(part 1 of 3)
# Autodesk Inventor assembly: HDR_2.54mm_RGB4078660_1
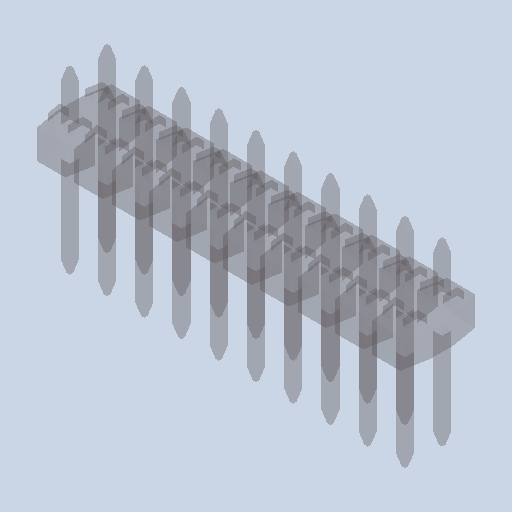
[picture p0: Inventor's stored thumbnail of the model, 512x512]
Saved by Autodesk Inventor 2026 (Build 300175050, 175E)
## iProperties
Created: 2025-07-29
Part Number: HDR_2.54mm_RGB4078660_1
Document SubType Name: Assembly
Designer: tdxt
Author: tdxt
## Documents named in this file (625)
- D:\Github\Pandoras_Box\CAD\pandoras_box_R2\pandoras_box_R2\HDR_2.54mm_RGB4078660_1.iam
- D:\Github\Pandoras_Box\CAD\pandoras_box_R2\pandoras_box_R2\Open CASCADE STEP translator 6.8 1.452.1.1.ipt
- D:\Github\Pandoras_Box\CAD\pandoras_box_R2\pandoras_box_R2\Open CASCADE STEP translator 6.8 1.452.1.2.ipt
- D:\Github\Pandoras_Box\CAD\pandoras_box_R2\pandoras_box_R2\Open CASCADE STEP translator 6.8 1.452.1.3.ipt
- D:\Github\Pandoras_Box\CAD\pandoras_box_R2\pandoras_box_R2\Open CASCADE STEP translator 6.8 1.452.1.4.ipt
- D:\Github\Pandoras_Box\CAD\pandoras_box_R2\pandoras_box_R2\Open CASCADE STEP translator 6.8 1.452.1.5.ipt
- D:\Github\Pandoras_Box\CAD\pandoras_box_R2\pandoras_box_R2\Open CASCADE STEP translator 6.8 1.452.1.6.ipt
- D:\Github\Pandoras_Box\CAD\pandoras_box_R2\pandoras_box_R2\Open CASCADE STEP translator 6.8 1.452.1.7.ipt
- D:\Github\Pandoras_Box\CAD\pandoras_box_R2\pandoras_box_R2\Open CASCADE STEP translator 6.8 1.452.1.8.ipt
- D:\Github\Pandoras_Box\CAD\pandoras_box_R2\pandoras_box_R2\Open CASCADE STEP translator 6.8 1.452.1.9.ipt
- D:\Github\Pandoras_Box\CAD\pandoras_box_R2\pandoras_box_R2\Open CASCADE STEP translator 6.8 1.452.1.10.ipt
- D:\Github\Pandoras_Box\CAD\pandoras_box_R2\pandoras_box_R2\Open CASCADE STEP translator 6.8 1.452.1.11.ipt
- D:\Github\Pandoras_Box\CAD\pandoras_box_R2\pandoras_box_R2\Open CASCADE STEP translator 6.8 1.452.1.12.ipt
- D:\Github\Pandoras_Box\CAD\pandoras_box_R2\pandoras_box_R2\Open CASCADE STEP translator 6.8 1.452.1.13.ipt
- D:\Github\Pandoras_Box\CAD\pandoras_box_R2\pandoras_box_R2\Open CASCADE STEP translator 6.8 1.452.1.14.ipt
- D:\Github\Pandoras_Box\CAD\pandoras_box_R2\pandoras_box_R2\Open CASCADE STEP translator 6.8 1.452.1.15.ipt
- D:\Github\Pandoras_Box\CAD\pandoras_box_R2\pandoras_box_R2\Open CASCADE STEP translator 6.8 1.452.1.16.ipt
- D:\Github\Pandoras_Box\CAD\pandoras_box_R2\pandoras_box_R2\Open CASCADE STEP translator 6.8 1.452.1.17.ipt
- D:\Github\Pandoras_Box\CAD\pandoras_box_R2\pandoras_box_R2\Open CASCADE STEP translator 6.8 1.452.1.18.ipt
- D:\Github\Pandoras_Box\CAD\pandoras_box_R2\pandoras_box_R2\Open CASCADE STEP translator 6.8 1.452.1.19.ipt
- D:\Github\Pandoras_Box\CAD\pandoras_box_R2\pandoras_box_R2\Open CASCADE STEP translator 6.8 1.452.1.20.ipt
- D:\Github\Pandoras_Box\CAD\pandoras_box_R2\pandoras_box_R2\Open CASCADE STEP translator 6.8 1.452.1.21.ipt
- D:\Github\Pandoras_Box\CAD\pandoras_box_R2\pandoras_box_R2\Open CASCADE STEP translator 6.8 1.452.1.22.ipt
- D:\Github\Pandoras_Box\CAD\pandoras_box_R2\pandoras_box_R2\Open CASCADE STEP translator 6.8 1.452.1.23.ipt
- D:\Github\Pandoras_Box\CAD\pandoras_box_R2\pandoras_box_R2\Open CASCADE STEP translator 6.8 1.452.1.24.ipt
- D:\Github\Pandoras_Box\CAD\pandoras_box_R2\pandoras_box_R2\Open CASCADE STEP translator 6.8 1.452.1.25.ipt
- D:\Github\Pandoras_Box\CAD\pandoras_box_R2\pandoras_box_R2\Open CASCADE STEP translator 6.8 1.452.1.26.ipt
- D:\Github\Pandoras_Box\CAD\pandoras_box_R2\pandoras_box_R2\Open CASCADE STEP translator 6.8 1.452.1.27.ipt
- D:\Github\Pandoras_Box\CAD\pandoras_box_R2\pandoras_box_R2\Open CASCADE STEP translator 6.8 1.452.1.28.ipt
- D:\Github\Pandoras_Box\CAD\pandoras_box_R2\pandoras_box_R2\Open CASCADE STEP translator 6.8 1.452.1.29.ipt
- D:\Github\Pandoras_Box\CAD\pandoras_box_R2\pandoras_box_R2\Open CASCADE STEP translator 6.8 1.452.1.30.ipt
- D:\Github\Pandoras_Box\CAD\pandoras_box_R2\pandoras_box_R2\Open CASCADE STEP translator 6.8 1.452.1.31.ipt
- D:\Github\Pandoras_Box\CAD\pandoras_box_R2\pandoras_box_R2\Open CASCADE STEP translator 6.8 1.452.1.32.ipt
- D:\Github\Pandoras_Box\CAD\pandoras_box_R2\pandoras_box_R2\Open CASCADE STEP translator 6.8 1.452.1.33.ipt
- D:\Github\Pandoras_Box\CAD\pandoras_box_R2\pandoras_box_R2\Open CASCADE STEP translator 6.8 1.452.1.34.ipt
- D:\Github\Pandoras_Box\CAD\pandoras_box_R2\pandoras_box_R2\Open CASCADE STEP translator 6.8 1.452.1.35.ipt
- D:\Github\Pandoras_Box\CAD\pandoras_box_R2\pandoras_box_R2\Open CASCADE STEP translator 6.8 1.452.1.36.ipt
- D:\Github\Pandoras_Box\CAD\pandoras_box_R2\pandoras_box_R2\Open CASCADE STEP translator 6.8 1.452.1.37.ipt
- D:\Github\Pandoras_Box\CAD\pandoras_box_R2\pandoras_box_R2\Open CASCADE STEP translator 6.8 1.452.1.38.ipt
- D:\Github\Pandoras_Box\CAD\pandoras_box_R2\pandoras_box_R2\Open CASCADE STEP translator 6.8 1.452.1.39.ipt
- D:\Github\Pandoras_Box\CAD\pandoras_box_R2\pandoras_box_R2\Open CASCADE STEP translator 6.8 1.452.1.40.ipt
- D:\Github\Pandoras_Box\CAD\pandoras_box_R2\pandoras_box_R2\Open CASCADE STEP translator 6.8 1.452.1.41.ipt
- D:\Github\Pandoras_Box\CAD\pandoras_box_R2\pandoras_box_R2\Open CASCADE STEP translator 6.8 1.452.1.42.ipt
- D:\Github\Pandoras_Box\CAD\pandoras_box_R2\pandoras_box_R2\Open CASCADE STEP translator 6.8 1.452.1.43.ipt
- D:\Github\Pandoras_Box\CAD\pandoras_box_R2\pandoras_box_R2\Open CASCADE STEP translator 6.8 1.452.1.44.ipt
- D:\Github\Pandoras_Box\CAD\pandoras_box_R2\pandoras_box_R2\Open CASCADE STEP translator 6.8 1.452.1.45.ipt
- D:\Github\Pandoras_Box\CAD\pandoras_box_R2\pandoras_box_R2\Open CASCADE STEP translator 6.8 1.452.1.46.ipt
- D:\Github\Pandoras_Box\CAD\pandoras_box_R2\pandoras_box_R2\Open CASCADE STEP translator 6.8 1.452.1.47.ipt
- D:\Github\Pandoras_Box\CAD\pandoras_box_R2\pandoras_box_R2\Open CASCADE STEP translator 6.8 1.452.1.48.ipt
- D:\Github\Pandoras_Box\CAD\pandoras_box_R2\pandoras_box_R2\Open CASCADE STEP translator 6.8 1.452.1.49.ipt
- D:\Github\Pandoras_Box\CAD\pandoras_box_R2\pandoras_box_R2\Open CASCADE STEP translator 6.8 1.452.1.50.ipt
- D:\Github\Pandoras_Box\CAD\pandoras_box_R2\pandoras_box_R2\Open CASCADE STEP translator 6.8 1.452.1.51.ipt
- D:\Github\Pandoras_Box\CAD\pandoras_box_R2\pandoras_box_R2\Open CASCADE STEP translator 6.8 1.452.1.52.ipt
- D:\Github\Pandoras_Box\CAD\pandoras_box_R2\pandoras_box_R2\Open CASCADE STEP translator 6.8 1.452.1.53.ipt
- D:\Github\Pandoras_Box\CAD\pandoras_box_R2\pandoras_box_R2\Open CASCADE STEP translator 6.8 1.452.1.54.ipt
- D:\Github\Pandoras_Box\CAD\pandoras_box_R2\pandoras_box_R2\Open CASCADE STEP translator 6.8 1.452.1.55.ipt
- D:\Github\Pandoras_Box\CAD\pandoras_box_R2\pandoras_box_R2\Open CASCADE STEP translator 6.8 1.452.1.56.ipt
- D:\Github\Pandoras_Box\CAD\pandoras_box_R2\pandoras_box_R2\Open CASCADE STEP translator 6.8 1.452.1.57.ipt
- D:\Github\Pandoras_Box\CAD\pandoras_box_R2\pandoras_box_R2\Open CASCADE STEP translator 6.8 1.452.1.58.ipt
- D:\Github\Pandoras_Box\CAD\pandoras_box_R2\pandoras_box_R2\Open CASCADE STEP translator 6.8 1.452.1.59.ipt
- D:\Github\Pandoras_Box\CAD\pandoras_box_R2\pandoras_box_R2\Open CASCADE STEP translator 6.8 1.452.1.60.ipt
- D:\Github\Pandoras_Box\CAD\pandoras_box_R2\pandoras_box_R2\Open CASCADE STEP translator 6.8 1.452.1.61.ipt
- D:\Github\Pandoras_Box\CAD\pandoras_box_R2\pandoras_box_R2\Open CASCADE STEP translator 6.8 1.452.1.62.ipt
- D:\Github\Pandoras_Box\CAD\pandoras_box_R2\pandoras_box_R2\Open CASCADE STEP translator 6.8 1.452.1.63.ipt
- D:\Github\Pandoras_Box\CAD\pandoras_box_R2\pandoras_box_R2\Open CASCADE STEP translator 6.8 1.452.1.64.ipt
- D:\Github\Pandoras_Box\CAD\pandoras_box_R2\pandoras_box_R2\Open CASCADE STEP translator 6.8 1.452.1.65.ipt
- D:\Github\Pandoras_Box\CAD\pandoras_box_R2\pandoras_box_R2\Open CASCADE STEP translator 6.8 1.452.1.66.ipt
- D:\Github\Pandoras_Box\CAD\pandoras_box_R2\pandoras_box_R2\Open CASCADE STEP translator 6.8 1.452.1.67.ipt
- D:\Github\Pandoras_Box\CAD\pandoras_box_R2\pandoras_box_R2\Open CASCADE STEP translator 6.8 1.452.1.68.ipt
- D:\Github\Pandoras_Box\CAD\pandoras_box_R2\pandoras_box_R2\Open CASCADE STEP translator 6.8 1.452.1.69.ipt
- D:\Github\Pandoras_Box\CAD\pandoras_box_R2\pandoras_box_R2\Open CASCADE STEP translator 6.8 1.452.1.70.ipt
- D:\Github\Pandoras_Box\CAD\pandoras_box_R2\pandoras_box_R2\Open CASCADE STEP translator 6.8 1.452.1.71.ipt
- D:\Github\Pandoras_Box\CAD\pandoras_box_R2\pandoras_box_R2\Open CASCADE STEP translator 6.8 1.452.1.72.ipt
- D:\Github\Pandoras_Box\CAD\pandoras_box_R2\pandoras_box_R2\Open CASCADE STEP translator 6.8 1.452.1.73.ipt
- D:\Github\Pandoras_Box\CAD\pandoras_box_R2\pandoras_box_R2\Open CASCADE STEP translator 6.8 1.452.1.74.ipt
- D:\Github\Pandoras_Box\CAD\pandoras_box_R2\pandoras_box_R2\Open CASCADE STEP translator 6.8 1.452.1.75.ipt
- D:\Github\Pandoras_Box\CAD\pandoras_box_R2\pandoras_box_R2\Open CASCADE STEP translator 6.8 1.452.1.76.ipt
- D:\Github\Pandoras_Box\CAD\pandoras_box_R2\pandoras_box_R2\Open CASCADE STEP translator 6.8 1.452.1.77.ipt
- D:\Github\Pandoras_Box\CAD\pandoras_box_R2\pandoras_box_R2\Open CASCADE STEP translator 6.8 1.452.1.78.ipt
- D:\Github\Pandoras_Box\CAD\pandoras_box_R2\pandoras_box_R2\Open CASCADE STEP translator 6.8 1.452.1.79.ipt
- D:\Github\Pandoras_Box\CAD\pandoras_box_R2\pandoras_box_R2\Open CASCADE STEP translator 6.8 1.452.1.80.ipt
- D:\Github\Pandoras_Box\CAD\pandoras_box_R2\pandoras_box_R2\Open CASCADE STEP translator 6.8 1.452.1.81.ipt
- D:\Github\Pandoras_Box\CAD\pandoras_box_R2\pandoras_box_R2\Open CASCADE STEP translator 6.8 1.452.1.82.ipt
- D:\Github\Pandoras_Box\CAD\pandoras_box_R2\pandoras_box_R2\Open CASCADE STEP translator 6.8 1.452.1.83.ipt
- D:\Github\Pandoras_Box\CAD\pandoras_box_R2\pandoras_box_R2\Open CASCADE STEP translator 6.8 1.452.1.84.ipt
- D:\Github\Pandoras_Box\CAD\pandoras_box_R2\pandoras_box_R2\Open CASCADE STEP translator 6.8 1.452.1.85.ipt
- D:\Github\Pandoras_Box\CAD\pandoras_box_R2\pandoras_box_R2\Open CASCADE STEP translator 6.8 1.452.1.86.ipt
- D:\Github\Pandoras_Box\CAD\pandoras_box_R2\pandoras_box_R2\Open CASCADE STEP translator 6.8 1.452.1.87.ipt
- D:\Github\Pandoras_Box\CAD\pandoras_box_R2\pandoras_box_R2\Open CASCADE STEP translator 6.8 1.452.1.88.ipt
- D:\Github\Pandoras_Box\CAD\pandoras_box_R2\pandoras_box_R2\Open CASCADE STEP translator 6.8 1.452.1.89.ipt
- D:\Github\Pandoras_Box\CAD\pandoras_box_R2\pandoras_box_R2\Open CASCADE STEP translator 6.8 1.452.1.90.ipt
- D:\Github\Pandoras_Box\CAD\pandoras_box_R2\pandoras_box_R2\Open CASCADE STEP translator 6.8 1.452.1.91.ipt
- D:\Github\Pandoras_Box\CAD\pandoras_box_R2\pandoras_box_R2\Open CASCADE STEP translator 6.8 1.452.1.92.ipt
- D:\Github\Pandoras_Box\CAD\pandoras_box_R2\pandoras_box_R2\Open CASCADE STEP translator 6.8 1.452.1.93.ipt
- D:\Github\Pandoras_Box\CAD\pandoras_box_R2\pandoras_box_R2\Open CASCADE STEP translator 6.8 1.452.1.94.ipt
- D:\Github\Pandoras_Box\CAD\pandoras_box_R2\pandoras_box_R2\Open CASCADE STEP translator 6.8 1.452.1.95.ipt
- D:\Github\Pandoras_Box\CAD\pandoras_box_R2\pandoras_box_R2\Open CASCADE STEP translator 6.8 1.452.1.96.ipt
- D:\Github\Pandoras_Box\CAD\pandoras_box_R2\pandoras_box_R2\Open CASCADE STEP translator 6.8 1.452.1.97.ipt
- D:\Github\Pandoras_Box\CAD\pandoras_box_R2\pandoras_box_R2\Open CASCADE STEP translator 6.8 1.452.1.98.ipt
- D:\Github\Pandoras_Box\CAD\pandoras_box_R2\pandoras_box_R2\Open CASCADE STEP translator 6.8 1.452.1.99.ipt
- D:\Github\Pandoras_Box\CAD\pandoras_box_R2\pandoras_box_R2\Open CASCADE STEP translator 6.8 1.452.1.100.ipt
- D:\Github\Pandoras_Box\CAD\pandoras_box_R2\pandoras_box_R2\Open CASCADE STEP translator 6.8 1.452.1.101.ipt
- D:\Github\Pandoras_Box\CAD\pandoras_box_R2\pandoras_box_R2\Open CASCADE STEP translator 6.8 1.452.1.102.ipt
- D:\Github\Pandoras_Box\CAD\pandoras_box_R2\pandoras_box_R2\Open CASCADE STEP translator 6.8 1.452.1.103.ipt
- D:\Github\Pandoras_Box\CAD\pandoras_box_R2\pandoras_box_R2\Open CASCADE STEP translator 6.8 1.452.1.104.ipt
- D:\Github\Pandoras_Box\CAD\pandoras_box_R2\pandoras_box_R2\Open CASCADE STEP translator 6.8 1.452.1.105.ipt
- D:\Github\Pandoras_Box\CAD\pandoras_box_R2\pandoras_box_R2\Open CASCADE STEP translator 6.8 1.452.1.106.ipt
- D:\Github\Pandoras_Box\CAD\pandoras_box_R2\pandoras_box_R2\Open CASCADE STEP translator 6.8 1.452.1.107.ipt
- D:\Github\Pandoras_Box\CAD\pandoras_box_R2\pandoras_box_R2\Open CASCADE STEP translator 6.8 1.452.1.108.ipt
- D:\Github\Pandoras_Box\CAD\pandoras_box_R2\pandoras_box_R2\Open CASCADE STEP translator 6.8 1.452.1.109.ipt
- D:\Github\Pandoras_Box\CAD\pandoras_box_R2\pandoras_box_R2\Open CASCADE STEP translator 6.8 1.452.1.110.ipt
- D:\Github\Pandoras_Box\CAD\pandoras_box_R2\pandoras_box_R2\Open CASCADE STEP translator 6.8 1.452.1.111.ipt
- D:\Github\Pandoras_Box\CAD\pandoras_box_R2\pandoras_box_R2\Open CASCADE STEP translator 6.8 1.452.1.112.ipt
- D:\Github\Pandoras_Box\CAD\pandoras_box_R2\pandoras_box_R2\Open CASCADE STEP translator 6.8 1.452.1.113.ipt
- D:\Github\Pandoras_Box\CAD\pandoras_box_R2\pandoras_box_R2\Open CASCADE STEP translator 6.8 1.452.1.114.ipt
- D:\Github\Pandoras_Box\CAD\pandoras_box_R2\pandoras_box_R2\Open CASCADE STEP translator 6.8 1.452.1.115.ipt
- D:\Github\Pandoras_Box\CAD\pandoras_box_R2\pandoras_box_R2\Open CASCADE STEP translator 6.8 1.452.1.116.ipt
- D:\Github\Pandoras_Box\CAD\pandoras_box_R2\pandoras_box_R2\Open CASCADE STEP translator 6.8 1.452.1.117.ipt
- D:\Github\Pandoras_Box\CAD\pandoras_box_R2\pandoras_box_R2\Open CASCADE STEP translator 6.8 1.452.1.118.ipt
- D:\Github\Pandoras_Box\CAD\pandoras_box_R2\pandoras_box_R2\Open CASCADE STEP translator 6.8 1.452.1.119.ipt
- D:\Github\Pandoras_Box\CAD\pandoras_box_R2\pandoras_box_R2\Open CASCADE STEP translator 6.8 1.452.1.120.ipt
- D:\Github\Pandoras_Box\CAD\pandoras_box_R2\pandoras_box_R2\Open CASCADE STEP translator 6.8 1.452.1.121.ipt
- D:\Github\Pandoras_Box\CAD\pandoras_box_R2\pandoras_box_R2\Open CASCADE STEP translator 6.8 1.452.1.122.ipt
- D:\Github\Pandoras_Box\CAD\pandoras_box_R2\pandoras_box_R2\Open CASCADE STEP translator 6.8 1.452.1.123.ipt
- D:\Github\Pandoras_Box\CAD\pandoras_box_R2\pandoras_box_R2\Open CASCADE STEP translator 6.8 1.452.1.124.ipt
- D:\Github\Pandoras_Box\CAD\pandoras_box_R2\pandoras_box_R2\Open CASCADE STEP translator 6.8 1.452.1.125.ipt
- D:\Github\Pandoras_Box\CAD\pandoras_box_R2\pandoras_box_R2\Open CASCADE STEP translator 6.8 1.452.1.126.ipt
- D:\Github\Pandoras_Box\CAD\pandoras_box_R2\pandoras_box_R2\Open CASCADE STEP translator 6.8 1.452.1.127.ipt
- D:\Github\Pandoras_Box\CAD\pandoras_box_R2\pandoras_box_R2\Open CASCADE STEP translator 6.8 1.452.1.128.ipt
- D:\Github\Pandoras_Box\CAD\pandoras_box_R2\pandoras_box_R2\Open CASCADE STEP translator 6.8 1.452.1.129.ipt
- D:\Github\Pandoras_Box\CAD\pandoras_box_R2\pandoras_box_R2\Open CASCADE STEP translator 6.8 1.452.1.130.ipt
- D:\Github\Pandoras_Box\CAD\pandoras_box_R2\pandoras_box_R2\Open CASCADE STEP translator 6.8 1.452.1.131.ipt
- D:\Github\Pandoras_Box\CAD\pandoras_box_R2\pandoras_box_R2\Open CASCADE STEP translator 6.8 1.452.1.132.ipt
- D:\Github\Pandoras_Box\CAD\pandoras_box_R2\pandoras_box_R2\Open CASCADE STEP translator 6.8 1.452.1.133.ipt
- D:\Github\Pandoras_Box\CAD\pandoras_box_R2\pandoras_box_R2\Open CASCADE STEP translator 6.8 1.452.1.134.ipt
- D:\Github\Pandoras_Box\CAD\pandoras_box_R2\pandoras_box_R2\Open CASCADE STEP translator 6.8 1.452.1.135.ipt
- D:\Github\Pandoras_Box\CAD\pandoras_box_R2\pandoras_box_R2\Open CASCADE STEP translator 6.8 1.452.1.136.ipt
- D:\Github\Pandoras_Box\CAD\pandoras_box_R2\pandoras_box_R2\Open CASCADE STEP translator 6.8 1.452.1.137.ipt
- D:\Github\Pandoras_Box\CAD\pandoras_box_R2\pandoras_box_R2\Open CASCADE STEP translator 6.8 1.452.1.138.ipt
- D:\Github\Pandoras_Box\CAD\pandoras_box_R2\pandoras_box_R2\Open CASCADE STEP translator 6.8 1.452.1.139.ipt
- D:\Github\Pandoras_Box\CAD\pandoras_box_R2\pandoras_box_R2\Open CASCADE STEP translator 6.8 1.452.1.140.ipt
- D:\Github\Pandoras_Box\CAD\pandoras_box_R2\pandoras_box_R2\Open CASCADE STEP translator 6.8 1.452.1.141.ipt
- D:\Github\Pandoras_Box\CAD\pandoras_box_R2\pandoras_box_R2\Open CASCADE STEP translator 6.8 1.452.1.142.ipt
- D:\Github\Pandoras_Box\CAD\pandoras_box_R2\pandoras_box_R2\Open CASCADE STEP translator 6.8 1.452.1.143.ipt
- D:\Github\Pandoras_Box\CAD\pandoras_box_R2\pandoras_box_R2\Open CASCADE STEP translator 6.8 1.452.1.144.ipt
- D:\Github\Pandoras_Box\CAD\pandoras_box_R2\pandoras_box_R2\Open CASCADE STEP translator 6.8 1.452.1.145.ipt
- D:\Github\Pandoras_Box\CAD\pandoras_box_R2\pandoras_box_R2\Open CASCADE STEP translator 6.8 1.452.1.146.ipt
- D:\Github\Pandoras_Box\CAD\pandoras_box_R2\pandoras_box_R2\Open CASCADE STEP translator 6.8 1.452.1.147.ipt
- D:\Github\Pandoras_Box\CAD\pandoras_box_R2\pandoras_box_R2\Open CASCADE STEP translator 6.8 1.452.1.148.ipt
- D:\Github\Pandoras_Box\CAD\pandoras_box_R2\pandoras_box_R2\Open CASCADE STEP translator 6.8 1.452.1.149.ipt
- D:\Github\Pandoras_Box\CAD\pandoras_box_R2\pandoras_box_R2\Open CASCADE STEP translator 6.8 1.452.1.150.ipt
- D:\Github\Pandoras_Box\CAD\pandoras_box_R2\pandoras_box_R2\Open CASCADE STEP translator 6.8 1.452.1.151.ipt
- D:\Github\Pandoras_Box\CAD\pandoras_box_R2\pandoras_box_R2\Open CASCADE STEP translator 6.8 1.452.1.152.ipt
- D:\Github\Pandoras_Box\CAD\pandoras_box_R2\pandoras_box_R2\Open CASCADE STEP translator 6.8 1.452.1.153.ipt
- D:\Github\Pandoras_Box\CAD\pandoras_box_R2\pandoras_box_R2\Open CASCADE STEP translator 6.8 1.452.1.154.ipt
- D:\Github\Pandoras_Box\CAD\pandoras_box_R2\pandoras_box_R2\Open CASCADE STEP translator 6.8 1.452.1.155.ipt
- D:\Github\Pandoras_Box\CAD\pandoras_box_R2\pandoras_box_R2\Open CASCADE STEP translator 6.8 1.452.1.156.ipt
- D:\Github\Pandoras_Box\CAD\pandoras_box_R2\pandoras_box_R2\Open CASCADE STEP translator 6.8 1.452.1.157.ipt
- D:\Github\Pandoras_Box\CAD\pandoras_box_R2\pandoras_box_R2\Open CASCADE STEP translator 6.8 1.452.1.158.ipt
- D:\Github\Pandoras_Box\CAD\pandoras_box_R2\pandoras_box_R2\Open CASCADE STEP translator 6.8 1.452.1.159.ipt
- D:\Github\Pandoras_Box\CAD\pandoras_box_R2\pandoras_box_R2\Open CASCADE STEP translator 6.8 1.452.1.160.ipt
- D:\Github\Pandoras_Box\CAD\pandoras_box_R2\pandoras_box_R2\Open CASCADE STEP translator 6.8 1.452.1.161.ipt
- D:\Github\Pandoras_Box\CAD\pandoras_box_R2\pandoras_box_R2\Open CASCADE STEP translator 6.8 1.452.1.162.ipt
- D:\Github\Pandoras_Box\CAD\pandoras_box_R2\pandoras_box_R2\Open CASCADE STEP translator 6.8 1.452.1.163.ipt
- D:\Github\Pandoras_Box\CAD\pandoras_box_R2\pandoras_box_R2\Open CASCADE STEP translator 6.8 1.452.1.164.ipt
- D:\Github\Pandoras_Box\CAD\pandoras_box_R2\pandoras_box_R2\Open CASCADE STEP translator 6.8 1.452.1.165.ipt
- D:\Github\Pandoras_Box\CAD\pandoras_box_R2\pandoras_box_R2\Open CASCADE STEP translator 6.8 1.452.1.166.ipt
- D:\Github\Pandoras_Box\CAD\pandoras_box_R2\pandoras_box_R2\Open CASCADE STEP translator 6.8 1.452.1.167.ipt
- D:\Github\Pandoras_Box\CAD\pandoras_box_R2\pandoras_box_R2\Open CASCADE STEP translator 6.8 1.452.1.168.ipt
- D:\Github\Pandoras_Box\CAD\pandoras_box_R2\pandoras_box_R2\Open CASCADE STEP translator 6.8 1.452.1.169.ipt
- D:\Github\Pandoras_Box\CAD\pandoras_box_R2\pandoras_box_R2\Open CASCADE STEP translator 6.8 1.452.1.170.ipt
- D:\Github\Pandoras_Box\CAD\pandoras_box_R2\pandoras_box_R2\Open CASCADE STEP translator 6.8 1.452.1.171.ipt
- D:\Github\Pandoras_Box\CAD\pandoras_box_R2\pandoras_box_R2\Open CASCADE STEP translator 6.8 1.452.1.172.ipt
- D:\Github\Pandoras_Box\CAD\pandoras_box_R2\pandoras_box_R2\Open CASCADE STEP translator 6.8 1.452.1.173.ipt
- D:\Github\Pandoras_Box\CAD\pandoras_box_R2\pandoras_box_R2\Open CASCADE STEP translator 6.8 1.452.1.174.ipt
- D:\Github\Pandoras_Box\CAD\pandoras_box_R2\pandoras_box_R2\Open CASCADE STEP translator 6.8 1.452.1.175.ipt
- D:\Github\Pandoras_Box\CAD\pandoras_box_R2\pandoras_box_R2\Open CASCADE STEP translator 6.8 1.452.1.176.ipt
- D:\Github\Pandoras_Box\CAD\pandoras_box_R2\pandoras_box_R2\Open CASCADE STEP translator 6.8 1.452.1.177.ipt
- D:\Github\Pandoras_Box\CAD\pandoras_box_R2\pandoras_box_R2\Open CASCADE STEP translator 6.8 1.452.1.178.ipt
- D:\Github\Pandoras_Box\CAD\pandoras_box_R2\pandoras_box_R2\Open CASCADE STEP translator 6.8 1.452.1.179.ipt
- D:\Github\Pandoras_Box\CAD\pandoras_box_R2\pandoras_box_R2\Open CASCADE STEP translator 6.8 1.452.1.180.ipt
- D:\Github\Pandoras_Box\CAD\pandoras_box_R2\pandoras_box_R2\Open CASCADE STEP translator 6.8 1.452.1.181.ipt
- D:\Github\Pandoras_Box\CAD\pandoras_box_R2\pandoras_box_R2\Open CASCADE STEP translator 6.8 1.452.1.182.ipt
- D:\Github\Pandoras_Box\CAD\pandoras_box_R2\pandoras_box_R2\Open CASCADE STEP translator 6.8 1.452.1.183.ipt
- D:\Github\Pandoras_Box\CAD\pandoras_box_R2\pandoras_box_R2\Open CASCADE STEP translator 6.8 1.452.1.184.ipt
- D:\Github\Pandoras_Box\CAD\pandoras_box_R2\pandoras_box_R2\Open CASCADE STEP translator 6.8 1.452.1.185.ipt
- D:\Github\Pandoras_Box\CAD\pandoras_box_R2\pandoras_box_R2\Open CASCADE STEP translator 6.8 1.452.1.186.ipt
- D:\Github\Pandoras_Box\CAD\pandoras_box_R2\pandoras_box_R2\Open CASCADE STEP translator 6.8 1.452.1.187.ipt
- D:\Github\Pandoras_Box\CAD\pandoras_box_R2\pandoras_box_R2\Open CASCADE STEP translator 6.8 1.452.1.188.ipt
- D:\Github\Pandoras_Box\CAD\pandoras_box_R2\pandoras_box_R2\Open CASCADE STEP translator 6.8 1.452.1.189.ipt
- D:\Github\Pandoras_Box\CAD\pandoras_box_R2\pandoras_box_R2\Open CASCADE STEP translator 6.8 1.452.1.190.ipt
- D:\Github\Pandoras_Box\CAD\pandoras_box_R2\pandoras_box_R2\Open CASCADE STEP translator 6.8 1.452.1.191.ipt
- D:\Github\Pandoras_Box\CAD\pandoras_box_R2\pandoras_box_R2\Open CASCADE STEP translator 6.8 1.452.1.192.ipt
- D:\Github\Pandoras_Box\CAD\pandoras_box_R2\pandoras_box_R2\Open CASCADE STEP translator 6.8 1.452.1.193.ipt
- D:\Github\Pandoras_Box\CAD\pandoras_box_R2\pandoras_box_R2\Open CASCADE STEP translator 6.8 1.452.1.194.ipt
- D:\Github\Pandoras_Box\CAD\pandoras_box_R2\pandoras_box_R2\Open CASCADE STEP translator 6.8 1.452.1.195.ipt
- D:\Github\Pandoras_Box\CAD\pandoras_box_R2\pandoras_box_R2\Open CASCADE STEP translator 6.8 1.452.1.196.ipt
- D:\Github\Pandoras_Box\CAD\pandoras_box_R2\pandoras_box_R2\Open CASCADE STEP translator 6.8 1.452.1.197.ipt
- D:\Github\Pandoras_Box\CAD\pandoras_box_R2\pandoras_box_R2\Open CASCADE STEP translator 6.8 1.452.1.198.ipt
- D:\Github\Pandoras_Box\CAD\pandoras_box_R2\pandoras_box_R2\Open CASCADE STEP translator 6.8 1.452.1.199.ipt
- D:\Github\Pandoras_Box\CAD\pandoras_box_R2\pandoras_box_R2\Open CASCADE STEP translator 6.8 1.452.1.200.ipt
- D:\Github\Pandoras_Box\CAD\pandoras_box_R2\pandoras_box_R2\Open CASCADE STEP translator 6.8 1.452.1.201.ipt
- D:\Github\Pandoras_Box\CAD\pandoras_box_R2\pandoras_box_R2\Open CASCADE STEP translator 6.8 1.452.1.202.ipt
- D:\Github\Pandoras_Box\CAD\pandoras_box_R2\pandoras_box_R2\Open CASCADE STEP translator 6.8 1.452.1.203.ipt
- D:\Github\Pandoras_Box\CAD\pandoras_box_R2\pandoras_box_R2\Open CASCADE STEP translator 6.8 1.452.1.204.ipt
- D:\Github\Pandoras_Box\CAD\pandoras_box_R2\pandoras_box_R2\Open CASCADE STEP translator 6.8 1.452.1.205.ipt
- D:\Github\Pandoras_Box\CAD\pandoras_box_R2\pandoras_box_R2\Open CASCADE STEP translator 6.8 1.452.1.206.ipt
- D:\Github\Pandoras_Box\CAD\pandoras_box_R2\pandoras_box_R2\Open CASCADE STEP translator 6.8 1.452.1.207.ipt
- D:\Github\Pandoras_Box\CAD\pandoras_box_R2\pandoras_box_R2\Open CASCADE STEP translator 6.8 1.452.1.208.ipt
- D:\Github\Pandoras_Box\CAD\pandoras_box_R2\pandoras_box_R2\Open CASCADE STEP translator 6.8 1.452.1.209.ipt
- D:\Github\Pandoras_Box\CAD\pandoras_box_R2\pandoras_box_R2\Open CASCADE STEP translator 6.8 1.452.1.210.ipt
- D:\Github\Pandoras_Box\CAD\pandoras_box_R2\pandoras_box_R2\Open CASCADE STEP translator 6.8 1.452.1.211.ipt
- D:\Github\Pandoras_Box\CAD\pandoras_box_R2\pandoras_box_R2\Open CASCADE STEP translator 6.8 1.452.1.212.ipt
- D:\Github\Pandoras_Box\CAD\pandoras_box_R2\pandoras_box_R2\Open CASCADE STEP translator 6.8 1.452.1.213.ipt
- D:\Github\Pandoras_Box\CAD\pandoras_box_R2\pandoras_box_R2\Open CASCADE STEP translator 6.8 1.452.1.214.ipt
- D:\Github\Pandoras_Box\CAD\pandoras_box_R2\pandoras_box_R2\Open CASCADE STEP translator 6.8 1.452.1.215.ipt
- D:\Github\Pandoras_Box\CAD\pandoras_box_R2\pandoras_box_R2\Open CASCADE STEP translator 6.8 1.452.1.216.ipt
- D:\Github\Pandoras_Box\CAD\pandoras_box_R2\pandoras_box_R2\Open CASCADE STEP translator 6.8 1.452.1.217.ipt
- D:\Github\Pandoras_Box\CAD\pandoras_box_R2\pandoras_box_R2\Open CASCADE STEP translator 6.8 1.452.1.218.ipt
- D:\Github\Pandoras_Box\CAD\pandoras_box_R2\pandoras_box_R2\Open CASCADE STEP translator 6.8 1.452.1.219.ipt
- D:\Github\Pandoras_Box\CAD\pandoras_box_R2\pandoras_box_R2\Open CASCADE STEP translator 6.8 1.452.1.220.ipt
- D:\Github\Pandoras_Box\CAD\pandoras_box_R2\pandoras_box_R2\Open CASCADE STEP translator 6.8 1.452.1.221.ipt
- D:\Github\Pandoras_Box\CAD\pandoras_box_R2\pandoras_box_R2\Open CASCADE STEP translator 6.8 1.452.1.222.ipt
- D:\Github\Pandoras_Box\CAD\pandoras_box_R2\pandoras_box_R2\Open CASCADE STEP translator 6.8 1.452.1.223.ipt
- D:\Github\Pandoras_Box\CAD\pandoras_box_R2\pandoras_box_R2\Open CASCADE STEP translator 6.8 1.452.1.224.ipt
- D:\Github\Pandoras_Box\CAD\pandoras_box_R2\pandoras_box_R2\Open CASCADE STEP translator 6.8 1.452.1.225.ipt
- D:\Github\Pandoras_Box\CAD\pandoras_box_R2\pandoras_box_R2\Open CASCADE STEP translator 6.8 1.452.1.226.ipt
- D:\Github\Pandoras_Box\CAD\pandoras_box_R2\pandoras_box_R2\Open CASCADE STEP translator 6.8 1.452.1.227.ipt
- D:\Github\Pandoras_Box\CAD\pandoras_box_R2\pandoras_box_R2\Open CASCADE STEP translator 6.8 1.452.1.228.ipt
- D:\Github\Pandoras_Box\CAD\pandoras_box_R2\pandoras_box_R2\Open CASCADE STEP translator 6.8 1.452.1.229.ipt
- D:\Github\Pandoras_Box\CAD\pandoras_box_R2\pandoras_box_R2\Open CASCADE STEP translator 6.8 1.452.1.230.ipt
- D:\Github\Pandoras_Box\CAD\pandoras_box_R2\pandoras_box_R2\Open CASCADE STEP translator 6.8 1.452.1.231.ipt
- D:\Github\Pandoras_Box\CAD\pandoras_box_R2\pandoras_box_R2\Open CASCADE STEP translator 6.8 1.452.1.232.ipt
- D:\Github\Pandoras_Box\CAD\pandoras_box_R2\pandoras_box_R2\Open CASCADE STEP translator 6.8 1.452.1.233.ipt
- D:\Github\Pandoras_Box\CAD\pandoras_box_R2\pandoras_box_R2\Open CASCADE STEP translator 6.8 1.452.1.234.ipt
- D:\Github\Pandoras_Box\CAD\pandoras_box_R2\pandoras_box_R2\Open CASCADE STEP translator 6.8 1.452.1.235.ipt
- D:\Github\Pandoras_Box\CAD\pandoras_box_R2\pandoras_box_R2\Open CASCADE STEP translator 6.8 1.452.1.236.ipt
- D:\Github\Pandoras_Box\CAD\pandoras_box_R2\pandoras_box_R2\Open CASCADE STEP translator 6.8 1.452.1.237.ipt
- D:\Github\Pandoras_Box\CAD\pandoras_box_R2\pandoras_box_R2\Open CASCADE STEP translator 6.8 1.452.1.238.ipt
- D:\Github\Pandoras_Box\CAD\pandoras_box_R2\pandoras_box_R2\Open CASCADE STEP translator 6.8 1.452.1.239.ipt
- D:\Github\Pandoras_Box\CAD\pandoras_box_R2\pandoras_box_R2\Open CASCADE STEP translator 6.8 1.452.1.240.ipt
- D:\Github\Pandoras_Box\CAD\pandoras_box_R2\pandoras_box_R2\Open CASCADE STEP translator 6.8 1.452.1.241.ipt
- D:\Github\Pandoras_Box\CAD\pandoras_box_R2\pandoras_box_R2\Open CASCADE STEP translator 6.8 1.452.1.242.ipt
- D:\Github\Pandoras_Box\CAD\pandoras_box_R2\pandoras_box_R2\Open CASCADE STEP translator 6.8 1.452.1.243.ipt
- D:\Github\Pandoras_Box\CAD\pandoras_box_R2\pandoras_box_R2\Open CASCADE STEP translator 6.8 1.452.1.244.ipt
- D:\Github\Pandoras_Box\CAD\pandoras_box_R2\pandoras_box_R2\Open CASCADE STEP translator 6.8 1.452.1.245.ipt
- D:\Github\Pandoras_Box\CAD\pandoras_box_R2\pandoras_box_R2\Open CASCADE STEP translator 6.8 1.452.1.246.ipt
- D:\Github\Pandoras_Box\CAD\pandoras_box_R2\pandoras_box_R2\Open CASCADE STEP translator 6.8 1.452.1.247.ipt
- D:\Github\Pandoras_Box\CAD\pandoras_box_R2\pandoras_box_R2\Open CASCADE STEP translator 6.8 1.452.1.248.ipt
- D:\Github\Pandoras_Box\CAD\pandoras_box_R2\pandoras_box_R2\Open CASCADE STEP translator 6.8 1.452.1.249.ipt
- D:\Github\Pandoras_Box\CAD\pandoras_box_R2\pandoras_box_R2\Open CASCADE STEP translator 6.8 1.452.1.250.ipt
- D:\Github\Pandoras_Box\CAD\pandoras_box_R2\pandoras_box_R2\Open CASCADE STEP translator 6.8 1.452.1.251.ipt
- D:\Github\Pandoras_Box\CAD\pandoras_box_R2\pandoras_box_R2\Open CASCADE STEP translator 6.8 1.452.1.252.ipt
- D:\Github\Pandoras_Box\CAD\pandoras_box_R2\pandoras_box_R2\Open CASCADE STEP translator 6.8 1.452.1.253.ipt
- D:\Github\Pandoras_Box\CAD\pandoras_box_R2\pandoras_box_R2\Open CASCADE STEP translator 6.8 1.452.1.254.ipt
- D:\Github\Pandoras_Box\CAD\pandoras_box_R2\pandoras_box_R2\Open CASCADE STEP translator 6.8 1.452.1.255.ipt
- D:\Github\Pandoras_Box\CAD\pandoras_box_R2\pandoras_box_R2\Open CASCADE STEP translator 6.8 1.452.1.256.ipt
- D:\Github\Pandoras_Box\CAD\pandoras_box_R2\pandoras_box_R2\Open CASCADE STEP translator 6.8 1.452.1.257.ipt
- D:\Github\Pandoras_Box\CAD\pandoras_box_R2\pandoras_box_R2\Open CASCADE STEP translator 6.8 1.452.1.258.ipt
- D:\Github\Pandoras_Box\CAD\pandoras_box_R2\pandoras_box_R2\Open CASCADE STEP translator 6.8 1.452.1.259.ipt
- D:\Github\Pandoras_Box\CAD\pandoras_box_R2\pandoras_box_R2\Open CASCADE STEP translator 6.8 1.452.1.260.ipt
- D:\Github\Pandoras_Box\CAD\pandoras_box_R2\pandoras_box_R2\Open CASCADE STEP translator 6.8 1.452.1.261.ipt
- D:\Github\Pandoras_Box\CAD\pandoras_box_R2\pandoras_box_R2\Open CASCADE STEP translator 6.8 1.452.1.262.ipt
- D:\Github\Pandoras_Box\CAD\pandoras_box_R2\pandoras_box_R2\Open CASCADE STEP translator 6.8 1.452.1.263.ipt
- D:\Github\Pandoras_Box\CAD\pandoras_box_R2\pandoras_box_R2\Open CASCADE STEP translator 6.8 1.452.1.264.ipt
- D:\Github\Pandoras_Box\CAD\pandoras_box_R2\pandoras_box_R2\Open CASCADE STEP translator 6.8 1.452.1.265.ipt
- D:\Github\Pandoras_Box\CAD\pandoras_box_R2\pandoras_box_R2\Open CASCADE STEP translator 6.8 1.452.1.266.ipt
- D:\Github\Pandoras_Box\CAD\pandoras_box_R2\pandoras_box_R2\Open CASCADE STEP translator 6.8 1.452.1.267.ipt
- D:\Github\Pandoras_Box\CAD\pandoras_box_R2\pandoras_box_R2\Open CASCADE STEP translator 6.8 1.452.1.268.ipt
- D:\Github\Pandoras_Box\CAD\pandoras_box_R2\pandoras_box_R2\Open CASCADE STEP translator 6.8 1.452.1.269.ipt
- D:\Github\Pandoras_Box\CAD\pandoras_box_R2\pandoras_box_R2\Open CASCADE STEP translator 6.8 1.452.1.270.ipt
- D:\Github\Pandoras_Box\CAD\pandoras_box_R2\pandoras_box_R2\Open CASCADE STEP translator 6.8 1.452.1.271.ipt
- D:\Github\Pandoras_Box\CAD\pandoras_box_R2\pandoras_box_R2\Open CASCADE STEP translator 6.8 1.452.1.272.ipt
- D:\Github\Pandoras_Box\CAD\pandoras_box_R2\pandoras_box_R2\Open CASCADE STEP translator 6.8 1.452.1.273.ipt
- D:\Github\Pandoras_Box\CAD\pandoras_box_R2\pandoras_box_R2\Open CASCADE STEP translator 6.8 1.452.1.274.ipt
- D:\Github\Pandoras_Box\CAD\pandoras_box_R2\pandoras_box_R2\Open CASCADE STEP translator 6.8 1.452.1.275.ipt
- D:\Github\Pandoras_Box\CAD\pandoras_box_R2\pandoras_box_R2\Open CASCADE STEP translator 6.8 1.452.1.276.ipt
- D:\Github\Pandoras_Box\CAD\pandoras_box_R2\pandoras_box_R2\Open CASCADE STEP translator 6.8 1.452.1.277.ipt
- D:\Github\Pandoras_Box\CAD\pandoras_box_R2\pandoras_box_R2\Open CASCADE STEP translator 6.8 1.452.1.278.ipt
- D:\Github\Pandoras_Box\CAD\pandoras_box_R2\pandoras_box_R2\Open CASCADE STEP translator 6.8 1.452.1.279.ipt
- D:\Github\Pandoras_Box\CAD\pandoras_box_R2\pandoras_box_R2\Open CASCADE STEP translator 6.8 1.452.1.280.ipt
- D:\Github\Pandoras_Box\CAD\pandoras_box_R2\pandoras_box_R2\Open CASCADE STEP translator 6.8 1.452.1.281.ipt
- D:\Github\Pandoras_Box\CAD\pandoras_box_R2\pandoras_box_R2\Open CASCADE STEP translator 6.8 1.452.1.282.ipt
- D:\Github\Pandoras_Box\CAD\pandoras_box_R2\pandoras_box_R2\Open CASCADE STEP translator 6.8 1.452.1.283.ipt
- D:\Github\Pandoras_Box\CAD\pandoras_box_R2\pandoras_box_R2\Open CASCADE STEP translator 6.8 1.452.1.284.ipt
- D:\Github\Pandoras_Box\CAD\pandoras_box_R2\pandoras_box_R2\Open CASCADE STEP translator 6.8 1.452.1.285.ipt
- D:\Github\Pandoras_Box\CAD\pandoras_box_R2\pandoras_box_R2\Open CASCADE STEP translator 6.8 1.452.1.286.ipt
- D:\Github\Pandoras_Box\CAD\pandoras_box_R2\pandoras_box_R2\Open CASCADE STEP translator 6.8 1.452.1.287.ipt
- D:\Github\Pandoras_Box\CAD\pandoras_box_R2\pandoras_box_R2\Open CASCADE STEP translator 6.8 1.452.1.288.ipt
- D:\Github\Pandoras_Box\CAD\pandoras_box_R2\pandoras_box_R2\Open CASCADE STEP translator 6.8 1.452.1.289.ipt
- D:\Github\Pandoras_Box\CAD\pandoras_box_R2\pandoras_box_R2\Open CASCADE STEP translator 6.8 1.452.1.290.ipt
- D:\Github\Pandoras_Box\CAD\pandoras_box_R2\pandoras_box_R2\Open CASCADE STEP translator 6.8 1.452.1.291.ipt
- D:\Github\Pandoras_Box\CAD\pandoras_box_R2\pandoras_box_R2\Open CASCADE STEP translator 6.8 1.452.1.292.ipt
- D:\Github\Pandoras_Box\CAD\pandoras_box_R2\pandoras_box_R2\Open CASCADE STEP translator 6.8 1.452.1.293.ipt
- D:\Github\Pandoras_Box\CAD\pandoras_box_R2\pandoras_box_R2\Open CASCADE STEP translator 6.8 1.452.1.294.ipt
- D:\Github\Pandoras_Box\CAD\pandoras_box_R2\pandoras_box_R2\Open CASCADE STEP translator 6.8 1.452.1.295.ipt
- D:\Github\Pandoras_Box\CAD\pandoras_box_R2\pandoras_box_R2\Open CASCADE STEP translator 6.8 1.452.1.296.ipt
- D:\Github\Pandoras_Box\CAD\pandoras_box_R2\pandoras_box_R2\Open CASCADE STEP translator 6.8 1.452.1.297.ipt
- D:\Github\Pandoras_Box\CAD\pandoras_box_R2\pandoras_box_R2\Open CASCADE STEP translator 6.8 1.452.1.298.ipt
- D:\Github\Pandoras_Box\CAD\pandoras_box_R2\pandoras_box_R2\Open CASCADE STEP translator 6.8 1.452.1.299.ipt
- D:\Github\Pandoras_Box\CAD\pandoras_box_R2\pandoras_box_R2\Open CASCADE STEP translator 6.8 1.452.1.300.ipt
- D:\Github\Pandoras_Box\CAD\pandoras_box_R2\pandoras_box_R2\Open CASCADE STEP translator 6.8 1.452.1.301.ipt
- D:\Github\Pandoras_Box\CAD\pandoras_box_R2\pandoras_box_R2\Open CASCADE STEP translator 6.8 1.452.1.302.ipt
- D:\Github\Pandoras_Box\CAD\pandoras_box_R2\pandoras_box_R2\Open CASCADE STEP translator 6.8 1.452.1.303.ipt
- D:\Github\Pandoras_Box\CAD\pandoras_box_R2\pandoras_box_R2\Open CASCADE STEP translator 6.8 1.452.1.304.ipt
- D:\Github\Pandoras_Box\CAD\pandoras_box_R2\pandoras_box_R2\Open CASCADE STEP translator 6.8 1.452.1.305.ipt
- D:\Github\Pandoras_Box\CAD\pandoras_box_R2\pandoras_box_R2\Open CASCADE STEP translator 6.8 1.452.1.306.ipt
- D:\Github\Pandoras_Box\CAD\pandoras_box_R2\pandoras_box_R2\Open CASCADE STEP translator 6.8 1.452.1.307.ipt
- D:\Github\Pandoras_Box\CAD\pandoras_box_R2\pandoras_box_R2\Open CASCADE STEP translator 6.8 1.452.1.308.ipt
- D:\Github\Pandoras_Box\CAD\pandoras_box_R2\pandoras_box_R2\Open CASCADE STEP translator 6.8 1.452.1.309.ipt
- D:\Github\Pandoras_Box\CAD\pandoras_box_R2\pandoras_box_R2\Open CASCADE STEP translator 6.8 1.452.1.310.ipt
- D:\Github\Pandoras_Box\CAD\pandoras_box_R2\pandoras_box_R2\Open CASCADE STEP translator 6.8 1.452.1.311.ipt
- D:\Github\Pandoras_Box\CAD\pandoras_box_R2\pandoras_box_R2\Open CASCADE STEP translator 6.8 1.452.1.312.ipt
- D:\Github\Pandoras_Box\CAD\pandoras_box_R2\pandoras_box_R2\Open CASCADE STEP translator 6.8 1.452.1.313.ipt
- D:\Github\Pandoras_Box\CAD\pandoras_box_R2\pandoras_box_R2\Open CASCADE STEP translator 6.8 1.452.1.314.ipt
- D:\Github\Pandoras_Box\CAD\pandoras_box_R2\pandoras_box_R2\Open CASCADE STEP translator 6.8 1.452.1.315.ipt
- D:\Github\Pandoras_Box\CAD\pandoras_box_R2\pandoras_box_R2\Open CASCADE STEP translator 6.8 1.452.1.316.ipt
- D:\Github\Pandoras_Box\CAD\pandoras_box_R2\pandoras_box_R2\Open CASCADE STEP translator 6.8 1.452.1.317.ipt
- D:\Github\Pandoras_Box\CAD\pandoras_box_R2\pandoras_box_R2\Open CASCADE STEP translator 6.8 1.452.1.318.ipt
- D:\Github\Pandoras_Box\CAD\pandoras_box_R2\pandoras_box_R2\Open CASCADE STEP translator 6.8 1.452.1.319.ipt
- D:\Github\Pandoras_Box\CAD\pandoras_box_R2\pandoras_box_R2\Open CASCADE STEP translator 6.8 1.452.1.320.ipt
- D:\Github\Pandoras_Box\CAD\pandoras_box_R2\pandoras_box_R2\Open CASCADE STEP translator 6.8 1.452.1.321.ipt
- D:\Github\Pandoras_Box\CAD\pandoras_box_R2\pandoras_box_R2\Open CASCADE STEP translator 6.8 1.452.1.322.ipt
- D:\Github\Pandoras_Box\CAD\pandoras_box_R2\pandoras_box_R2\Open CASCADE STEP translator 6.8 1.452.1.323.ipt
- D:\Github\Pandoras_Box\CAD\pandoras_box_R2\pandoras_box_R2\Open CASCADE STEP translator 6.8 1.452.1.324.ipt
- D:\Github\Pandoras_Box\CAD\pandoras_box_R2\pandoras_box_R2\Open CASCADE STEP translator 6.8 1.452.1.325.ipt
- D:\Github\Pandoras_Box\CAD\pandoras_box_R2\pandoras_box_R2\Open CASCADE STEP translator 6.8 1.452.1.326.ipt
- D:\Github\Pandoras_Box\CAD\pandoras_box_R2\pandoras_box_R2\Open CASCADE STEP translator 6.8 1.452.1.327.ipt
- D:\Github\Pandoras_Box\CAD\pandoras_box_R2\pandoras_box_R2\Open CASCADE STEP translator 6.8 1.452.1.328.ipt
- D:\Github\Pandoras_Box\CAD\pandoras_box_R2\pandoras_box_R2\Open CASCADE STEP translator 6.8 1.452.1.329.ipt
- D:\Github\Pandoras_Box\CAD\pandoras_box_R2\pandoras_box_R2\Open CASCADE STEP translator 6.8 1.452.1.330.ipt
- D:\Github\Pandoras_Box\CAD\pandoras_box_R2\pandoras_box_R2\Open CASCADE STEP translator 6.8 1.452.1.331.ipt
- D:\Github\Pandoras_Box\CAD\pandoras_box_R2\pandoras_box_R2\Open CASCADE STEP translator 6.8 1.452.1.332.ipt
- D:\Github\Pandoras_Box\CAD\pandoras_box_R2\pandoras_box_R2\Open CASCADE STEP translator 6.8 1.452.1.333.ipt
- D:\Github\Pandoras_Box\CAD\pandoras_box_R2\pandoras_box_R2\Open CASCADE STEP translator 6.8 1.452.1.334.ipt
- D:\Github\Pandoras_Box\CAD\pandoras_box_R2\pandoras_box_R2\Open CASCADE STEP translator 6.8 1.452.1.335.ipt
- D:\Github\Pandoras_Box\CAD\pandoras_box_R2\pandoras_box_R2\Open CASCADE STEP translator 6.8 1.452.1.336.ipt
- D:\Github\Pandoras_Box\CAD\pandoras_box_R2\pandoras_box_R2\Open CASCADE STEP translator 6.8 1.452.1.337.ipt
- D:\Github\Pandoras_Box\CAD\pandoras_box_R2\pandoras_box_R2\Open CASCADE STEP translator 6.8 1.452.1.338.ipt
- D:\Github\Pandoras_Box\CAD\pandoras_box_R2\pandoras_box_R2\Open CASCADE STEP translator 6.8 1.452.1.339.ipt
- D:\Github\Pandoras_Box\CAD\pandoras_box_R2\pandoras_box_R2\Open CASCADE STEP translator 6.8 1.452.1.340.ipt
- D:\Github\Pandoras_Box\CAD\pandoras_box_R2\pandoras_box_R2\Open CASCADE STEP translator 6.8 1.452.1.341.ipt
- D:\Github\Pandoras_Box\CAD\pandoras_box_R2\pandoras_box_R2\Open CASCADE STEP translator 6.8 1.452.1.342.ipt
- D:\Github\Pandoras_Box\CAD\pandoras_box_R2\pandoras_box_R2\Open CASCADE STEP translator 6.8 1.452.1.343.ipt
- D:\Github\Pandoras_Box\CAD\pandoras_box_R2\pandoras_box_R2\Open CASCADE STEP translator 6.8 1.452.1.344.ipt
- D:\Github\Pandoras_Box\CAD\pandoras_box_R2\pandoras_box_R2\Open CASCADE STEP translator 6.8 1.452.1.345.ipt
- D:\Github\Pandoras_Box\CAD\pandoras_box_R2\pandoras_box_R2\Open CASCADE STEP translator 6.8 1.452.1.346.ipt
- D:\Github\Pandoras_Box\CAD\pandoras_box_R2\pandoras_box_R2\Open CASCADE STEP translator 6.8 1.452.1.347.ipt
- D:\Github\Pandoras_Box\CAD\pandoras_box_R2\pandoras_box_R2\Open CASCADE STEP translator 6.8 1.452.1.348.ipt
- D:\Github\Pandoras_Box\CAD\pandoras_box_R2\pandoras_box_R2\Open CASCADE STEP translator 6.8 1.452.1.349.ipt
- D:\Github\Pandoras_Box\CAD\pandoras_box_R2\pandoras_box_R2\Open CASCADE STEP translator 6.8 1.452.1.350.ipt
- D:\Github\Pandoras_Box\CAD\pandoras_box_R2\pandoras_box_R2\Open CASCADE STEP translator 6.8 1.452.1.351.ipt
- D:\Github\Pandoras_Box\CAD\pandoras_box_R2\pandoras_box_R2\Open CASCADE STEP translator 6.8 1.452.1.352.ipt
- D:\Github\Pandoras_Box\CAD\pandoras_box_R2\pandoras_box_R2\Open CASCADE STEP translator 6.8 1.452.1.353.ipt
- D:\Github\Pandoras_Box\CAD\pandoras_box_R2\pandoras_box_R2\Open CASCADE STEP translator 6.8 1.452.1.354.ipt
- D:\Github\Pandoras_Box\CAD\pandoras_box_R2\pandoras_box_R2\Open CASCADE STEP translator 6.8 1.452.1.355.ipt
- D:\Github\Pandoras_Box\CAD\pandoras_box_R2\pandoras_box_R2\Open CASCADE STEP translator 6.8 1.452.1.356.ipt
- D:\Github\Pandoras_Box\CAD\pandoras_box_R2\pandoras_box_R2\Open CASCADE STEP translator 6.8 1.452.1.357.ipt
- D:\Github\Pandoras_Box\CAD\pandoras_box_R2\pandoras_box_R2\Open CASCADE STEP translator 6.8 1.452.1.358.ipt
- D:\Github\Pandoras_Box\CAD\pandoras_box_R2\pandoras_box_R2\Open CASCADE STEP translator 6.8 1.452.1.359.ipt
- D:\Github\Pandoras_Box\CAD\pandoras_box_R2\pandoras_box_R2\Open CASCADE STEP translator 6.8 1.452.1.360.ipt
- D:\Github\Pandoras_Box\CAD\pandoras_box_R2\pandoras_box_R2\Open CASCADE STEP translator 6.8 1.452.1.361.ipt
- D:\Github\Pandoras_Box\CAD\pandoras_box_R2\pandoras_box_R2\Open CASCADE STEP translator 6.8 1.452.1.362.ipt
- D:\Github\Pandoras_Box\CAD\pandoras_box_R2\pandoras_box_R2\Open CASCADE STEP translator 6.8 1.452.1.363.ipt
- D:\Github\Pandoras_Box\CAD\pandoras_box_R2\pandoras_box_R2\Open CASCADE STEP translator 6.8 1.452.1.364.ipt
- D:\Github\Pandoras_Box\CAD\pandoras_box_R2\pandoras_box_R2\Open CASCADE STEP translator 6.8 1.452.1.365.ipt
- D:\Github\Pandoras_Box\CAD\pandoras_box_R2\pandoras_box_R2\Open CASCADE STEP translator 6.8 1.452.1.366.ipt
- D:\Github\Pandoras_Box\CAD\pandoras_box_R2\pandoras_box_R2\Open CASCADE STEP translator 6.8 1.452.1.367.ipt
- D:\Github\Pandoras_Box\CAD\pandoras_box_R2\pandoras_box_R2\Open CASCADE STEP translator 6.8 1.452.1.368.ipt
- D:\Github\Pandoras_Box\CAD\pandoras_box_R2\pandoras_box_R2\Open CASCADE STEP translator 6.8 1.452.1.369.ipt
- D:\Github\Pandoras_Box\CAD\pandoras_box_R2\pandoras_box_R2\Open CASCADE STEP translator 6.8 1.452.1.370.ipt
- D:\Github\Pandoras_Box\CAD\pandoras_box_R2\pandoras_box_R2\Open CASCADE STEP translator 6.8 1.452.1.371.ipt
- D:\Github\Pandoras_Box\CAD\pandoras_box_R2\pandoras_box_R2\Open CASCADE STEP translator 6.8 1.452.1.372.ipt
- D:\Github\Pandoras_Box\CAD\pandoras_box_R2\pandoras_box_R2\Open CASCADE STEP translator 6.8 1.452.1.373.ipt
- D:\Github\Pandoras_Box\CAD\pandoras_box_R2\pandoras_box_R2\Open CASCADE STEP translator 6.8 1.452.1.374.ipt
- D:\Github\Pandoras_Box\CAD\pandoras_box_R2\pandoras_box_R2\Open CASCADE STEP translator 6.8 1.452.1.375.ipt
- D:\Github\Pandoras_Box\CAD\pandoras_box_R2\pandoras_box_R2\Open CASCADE STEP translator 6.8 1.452.1.376.ipt
- D:\Github\Pandoras_Box\CAD\pandoras_box_R2\pandoras_box_R2\Open CASCADE STEP translator 6.8 1.452.1.377.ipt
- D:\Github\Pandoras_Box\CAD\pandoras_box_R2\pandoras_box_R2\Open CASCADE STEP translator 6.8 1.452.1.378.ipt
- D:\Github\Pandoras_Box\CAD\pandoras_box_R2\pandoras_box_R2\Open CASCADE STEP translator 6.8 1.452.1.379.ipt
- D:\Github\Pandoras_Box\CAD\pandoras_box_R2\pandoras_box_R2\Open CASCADE STEP translator 6.8 1.452.1.380.ipt
- D:\Github\Pandoras_Box\CAD\pandoras_box_R2\pandoras_box_R2\Open CASCADE STEP translator 6.8 1.452.1.381.ipt
- D:\Github\Pandoras_Box\CAD\pandoras_box_R2\pandoras_box_R2\Open CASCADE STEP translator 6.8 1.452.1.382.ipt
- D:\Github\Pandoras_Box\CAD\pandoras_box_R2\pandoras_box_R2\Open CASCADE STEP translator 6.8 1.452.1.383.ipt
- D:\Github\Pandoras_Box\CAD\pandoras_box_R2\pandoras_box_R2\Open CASCADE STEP translator 6.8 1.452.1.384.ipt
- D:\Github\Pandoras_Box\CAD\pandoras_box_R2\pandoras_box_R2\Open CASCADE STEP translator 6.8 1.452.1.385.ipt
- D:\Github\Pandoras_Box\CAD\pandoras_box_R2\pandoras_box_R2\Open CASCADE STEP translator 6.8 1.452.1.386.ipt
- D:\Github\Pandoras_Box\CAD\pandoras_box_R2\pandoras_box_R2\Open CASCADE STEP translator 6.8 1.452.1.387.ipt
- D:\Github\Pandoras_Box\CAD\pandoras_box_R2\pandoras_box_R2\Open CASCADE STEP translator 6.8 1.452.1.388.ipt
- D:\Github\Pandoras_Box\CAD\pandoras_box_R2\pandoras_box_R2\Open CASCADE STEP translator 6.8 1.452.1.389.ipt
- D:\Github\Pandoras_Box\CAD\pandoras_box_R2\pandoras_box_R2\Open CASCADE STEP translator 6.8 1.452.1.390.ipt
- D:\Github\Pandoras_Box\CAD\pandoras_box_R2\pandoras_box_R2\Open CASCADE STEP translator 6.8 1.452.1.391.ipt
- D:\Github\Pandoras_Box\CAD\pandoras_box_R2\pandoras_box_R2\Open CASCADE STEP translator 6.8 1.452.1.392.ipt
- D:\Github\Pandoras_Box\CAD\pandoras_box_R2\pandoras_box_R2\Open CASCADE STEP translator 6.8 1.452.1.393.ipt
- D:\Github\Pandoras_Box\CAD\pandoras_box_R2\pandoras_box_R2\Open CASCADE STEP translator 6.8 1.452.1.394.ipt
- D:\Github\Pandoras_Box\CAD\pandoras_box_R2\pandoras_box_R2\Open CASCADE STEP translator 6.8 1.452.1.395.ipt
- D:\Github\Pandoras_Box\CAD\pandoras_box_R2\pandoras_box_R2\Open CASCADE STEP translator 6.8 1.452.1.396.ipt
- D:\Github\Pandoras_Box\CAD\pandoras_box_R2\pandoras_box_R2\Open CASCADE STEP translator 6.8 1.452.1.397.ipt
- D:\Github\Pandoras_Box\CAD\pandoras_box_R2\pandoras_box_R2\Open CASCADE STEP translator 6.8 1.452.1.398.ipt
- D:\Github\Pandoras_Box\CAD\pandoras_box_R2\pandoras_box_R2\Open CASCADE STEP translator 6.8 1.452.1.399.ipt
- D:\Github\Pandoras_Box\CAD\pandoras_box_R2\pandoras_box_R2\Open CASCADE STEP translator 6.8 1.452.1.400.ipt
- D:\Github\Pandoras_Box\CAD\pandoras_box_R2\pandoras_box_R2\Open CASCADE STEP translator 6.8 1.452.1.401.ipt
- D:\Github\Pandoras_Box\CAD\pandoras_box_R2\pandoras_box_R2\Open CASCADE STEP translator 6.8 1.452.1.402.ipt
- D:\Github\Pandoras_Box\CAD\pandoras_box_R2\pandoras_box_R2\Open CASCADE STEP translator 6.8 1.452.1.403.ipt
- D:\Github\Pandoras_Box\CAD\pandoras_box_R2\pandoras_box_R2\Open CASCADE STEP translator 6.8 1.452.1.404.ipt
- D:\Github\Pandoras_Box\CAD\pandoras_box_R2\pandoras_box_R2\Open CASCADE STEP translator 6.8 1.452.1.405.ipt
- D:\Github\Pandoras_Box\CAD\pandoras_box_R2\pandoras_box_R2\Open CASCADE STEP translator 6.8 1.452.1.406.ipt
- D:\Github\Pandoras_Box\CAD\pandoras_box_R2\pandoras_box_R2\Open CASCADE STEP translator 6.8 1.452.1.407.ipt
- D:\Github\Pandoras_Box\CAD\pandoras_box_R2\pandoras_box_R2\Open CASCADE STEP translator 6.8 1.452.1.408.ipt
- D:\Github\Pandoras_Box\CAD\pandoras_box_R2\pandoras_box_R2\Open CASCADE STEP translator 6.8 1.452.1.409.ipt
- D:\Github\Pandoras_Box\CAD\pandoras_box_R2\pandoras_box_R2\Open CASCADE STEP translator 6.8 1.452.1.410.ipt
- D:\Github\Pandoras_Box\CAD\pandoras_box_R2\pandoras_box_R2\Open CASCADE STEP translator 6.8 1.452.1.411.ipt
- D:\Github\Pandoras_Box\CAD\pandoras_box_R2\pandoras_box_R2\Open CASCADE STEP translator 6.8 1.452.1.412.ipt
- D:\Github\Pandoras_Box\CAD\pandoras_box_R2\pandoras_box_R2\Open CASCADE STEP translator 6.8 1.452.1.413.ipt
- D:\Github\Pandoras_Box\CAD\pandoras_box_R2\pandoras_box_R2\Open CASCADE STEP translator 6.8 1.452.1.414.ipt
- D:\Github\Pandoras_Box\CAD\pandoras_box_R2\pandoras_box_R2\Open CASCADE STEP translator 6.8 1.452.1.415.ipt
- D:\Github\Pandoras_Box\CAD\pandoras_box_R2\pandoras_box_R2\Open CASCADE STEP translator 6.8 1.452.1.416.ipt
- D:\Github\Pandoras_Box\CAD\pandoras_box_R2\pandoras_box_R2\Open CASCADE STEP translator 6.8 1.452.1.417.ipt
- D:\Github\Pandoras_Box\CAD\pandoras_box_R2\pandoras_box_R2\Open CASCADE STEP translator 6.8 1.452.1.418.ipt
- D:\Github\Pandoras_Box\CAD\pandoras_box_R2\pandoras_box_R2\Open CASCADE STEP translator 6.8 1.452.1.419.ipt
- D:\Github\Pandoras_Box\CAD\pandoras_box_R2\pandoras_box_R2\Open CASCADE STEP translator 6.8 1.452.1.420.ipt
- D:\Github\Pandoras_Box\CAD\pandoras_box_R2\pandoras_box_R2\Open CASCADE STEP translator 6.8 1.452.1.421.ipt
- D:\Github\Pandoras_Box\CAD\pandoras_box_R2\pandoras_box_R2\Open CASCADE STEP translator 6.8 1.452.1.422.ipt
- D:\Github\Pandoras_Box\CAD\pandoras_box_R2\pandoras_box_R2\Open CASCADE STEP translator 6.8 1.452.1.423.ipt
- D:\Github\Pandoras_Box\CAD\pandoras_box_R2\pandoras_box_R2\Open CASCADE STEP translator 6.8 1.452.1.424.ipt
- D:\Github\Pandoras_Box\CAD\pandoras_box_R2\pandoras_box_R2\Open CASCADE STEP translator 6.8 1.452.1.425.ipt
- D:\Github\Pandoras_Box\CAD\pandoras_box_R2\pandoras_box_R2\Open CASCADE STEP translator 6.8 1.452.1.426.ipt
- D:\Github\Pandoras_Box\CAD\pandoras_box_R2\pandoras_box_R2\Open CASCADE STEP translator 6.8 1.452.1.427.ipt
- D:\Github\Pandoras_Box\CAD\pandoras_box_R2\pandoras_box_R2\Open CASCADE STEP translator 6.8 1.452.1.428.ipt
- D:\Github\Pandoras_Box\CAD\pandoras_box_R2\pandoras_box_R2\Open CASCADE STEP translator 6.8 1.452.1.429.ipt
- D:\Github\Pandoras_Box\CAD\pandoras_box_R2\pandoras_box_R2\Open CASCADE STEP translator 6.8 1.452.1.430.ipt
- D:\Github\Pandoras_Box\CAD\pandoras_box_R2\pandoras_box_R2\Open CASCADE STEP translator 6.8 1.452.1.431.ipt
- D:\Github\Pandoras_Box\CAD\pandoras_box_R2\pandoras_box_R2\Open CASCADE STEP translator 6.8 1.452.1.432.ipt
- D:\Github\Pandoras_Box\CAD\pandoras_box_R2\pandoras_box_R2\Open CASCADE STEP translator 6.8 1.452.1.433.ipt
- D:\Github\Pandoras_Box\CAD\pandoras_box_R2\pandoras_box_R2\Open CASCADE STEP translator 6.8 1.452.1.434.ipt
- D:\Github\Pandoras_Box\CAD\pandoras_box_R2\pandoras_box_R2\Open CASCADE STEP translator 6.8 1.452.1.435.ipt
- D:\Github\Pandoras_Box\CAD\pandoras_box_R2\pandoras_box_R2\Open CASCADE STEP translator 6.8 1.452.1.436.ipt
- D:\Github\Pandoras_Box\CAD\pandoras_box_R2\pandoras_box_R2\Open CASCADE STEP translator 6.8 1.452.1.437.ipt
- D:\Github\Pandoras_Box\CAD\pandoras_box_R2\pandoras_box_R2\Open CASCADE STEP translator 6.8 1.452.1.438.ipt
- D:\Github\Pandoras_Box\CAD\pandoras_box_R2\pandoras_box_R2\Open CASCADE STEP translator 6.8 1.452.1.439.ipt
- D:\Github\Pandoras_Box\CAD\pandoras_box_R2\pandoras_box_R2\Open CASCADE STEP translator 6.8 1.452.1.440.ipt
- D:\Github\Pandoras_Box\CAD\pandoras_box_R2\pandoras_box_R2\Open CASCADE STEP translator 6.8 1.452.1.441.ipt
- D:\Github\Pandoras_Box\CAD\pandoras_box_R2\pandoras_box_R2\Open CASCADE STEP translator 6.8 1.452.1.442.ipt
- D:\Github\Pandoras_Box\CAD\pandoras_box_R2\pandoras_box_R2\Open CASCADE STEP translator 6.8 1.452.1.443.ipt
- D:\Github\Pandoras_Box\CAD\pandoras_box_R2\pandoras_box_R2\Open CASCADE STEP translator 6.8 1.452.1.444.ipt
- D:\Github\Pandoras_Box\CAD\pandoras_box_R2\pandoras_box_R2\Open CASCADE STEP translator 6.8 1.452.1.445.ipt
- D:\Github\Pandoras_Box\CAD\pandoras_box_R2\pandoras_box_R2\Open CASCADE STEP translator 6.8 1.452.1.446.ipt
- D:\Github\Pandoras_Box\CAD\pandoras_box_R2\pandoras_box_R2\Open CASCADE STEP translator 6.8 1.452.1.447.ipt
- D:\Github\Pandoras_Box\CAD\pandoras_box_R2\pandoras_box_R2\Open CASCADE STEP translator 6.8 1.452.1.448.ipt
- D:\Github\Pandoras_Box\CAD\pandoras_box_R2\pandoras_box_R2\Open CASCADE STEP translator 6.8 1.452.1.449.ipt